# Autodesk Inventor assembly: 主动轮锥齿轮
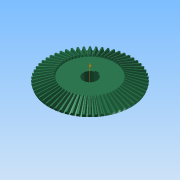
[picture p0: Inventor's stored thumbnail of the model, 180x180]
Saved by Autodesk Inventor 2015 (Build 190159000, 159)
## iProperties
Created: 2017-06-08
Part Number: 主动轮锥齿轮
Document SubType Name: Assembly
Designer: Administrator
Author: Administrator
## Documents named in this file (3)
- C:\Users\Administrator\Desktop\毕设改\主动轮锥齿轮.iam
- C:\Users\Administrator\Desktop\毕设改\主动轮锥齿轮\设计加速器\主动轮锥齿轮1.iam
- C:\Users\Administrator\Desktop\毕设改\主动轮锥齿轮配件.ipt
## Components (2 placed, 2 different names)
1. 主动轮锥齿轮:1 [sub-assembly] — 刚性:1
2. 主动轮锥齿轮配件:1 — 刚性:1
## Relationships (1: WeldJoint 1)
- 刚性:1 [WeldJoint]: 主动轮锥齿轮:1 ↔ 主动轮锥齿轮配件:1
